# Autodesk Inventor assembly: Coupler
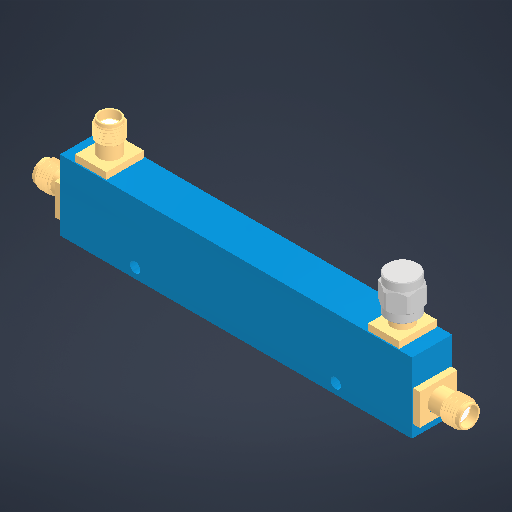
[picture p0: Inventor's stored thumbnail of the model, 512x512]
Saved by Autodesk Inventor 2026.2 (Build 302298010, 298A)
## iProperties
Created: 2026-06-11
Part Number: Coupler
Document SubType Name: Assembly
Designer: sonata
Author: sonata
## Documents named in this file (4)
- Z:\crush\Coupler.iam
- Z:\crush\Coupler.ipt
- Z:\crush\crush\sma-female-pcb-edge-launch-connector-031-pcb-thickness-1.snapshot.1\2985-6037\2985-6037\2985-6037.ipt
- Z:\crush\crush\185187850-9-70551432\70551432.ipt
## Components (6 placed, 3 different names)
1. Coupler:1 — Mate:1, Flush:1, Flush:2, Mate:2, Flush:3, Flush:4, Mate:3, Flush:5, Flush:6, Mate:4, Flush:7, Flush:8
2. 2985-6037:1 — Mate:1, Flush:1, Flush:2
3. 2985-6037:2 — Mate:2, Flush:3, Flush:4
4. 2985-6037:3 — Mate:4, Flush:7, Mate:5
5. 2985-6037:4 — Mate:3, Flush:5, Flush:6, Mate:5, Mate:6
6. 70551432:1 — Flush:8, Mate:6
## Relationships (14: Flush 8, Mate 6)
- Mate:1: Coupler:1 ↔ 2985-6037:1
- Flush:1 (0.3175 mm): Coupler:1 ↔ 2985-6037:1
- Flush:2 (3.0226 mm): Coupler:1 ↔ 2985-6037:1
- Mate:2: Coupler:1 ↔ 2985-6037:2
- Flush:3 (0.3175 mm): Coupler:1 ↔ 2985-6037:2
- Flush:4 (3.0226 mm): Coupler:1 ↔ 2985-6037:2
- Mate:3: Coupler:1 ↔ 2985-6037:4
- Flush:5 (0.3175 mm): Coupler:1 ↔ 2985-6037:4
- Flush:6 (3.5306 mm): Coupler:1 ↔ 2985-6037:4
- Mate:4: Coupler:1 ↔ 2985-6037:3
- Flush:7 (0.3175 mm): Coupler:1 ↔ 2985-6037:3
- Mate:5 (74.168 mm): 2985-6037:3 ↔ 2985-6037:4
- Flush:8 (-12.7 mm): Coupler:1 ↔ 70551432:1
- Mate:6: 2985-6037:4 ↔ 70551432:1
